# Autodesk Inventor assembly: center_4p_female
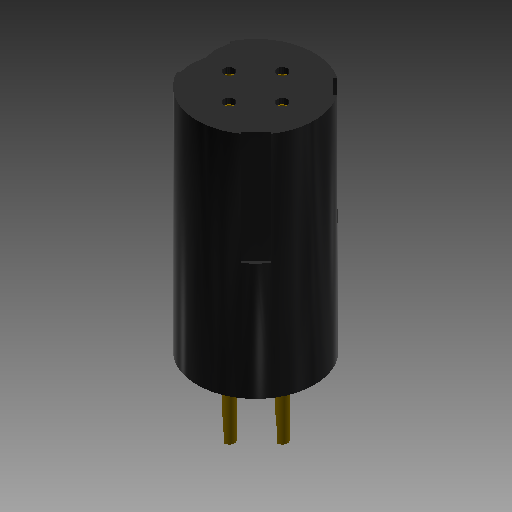
[picture p0: Inventor's stored thumbnail of the model, 512x512]
Saved by Autodesk Inventor 2018 (Build 220112000, 112)
## iProperties
Created: 2019-04-17
Part Number: center_4p_female
Document SubType Name: Assembly
Designer: ZEUSLAP
Author: ZEUSLAP
## Documents named in this file (3)
- C:\Users\ZEUSLAP\YandexDisk\Inventor\SP16 waterproof connector\parts\center_4p_female.iam
- C:\Users\ZEUSLAP\YandexDisk\Inventor\SP16 waterproof connector\parts\center_4p_female_body.ipt
- C:\Users\ZEUSLAP\YandexDisk\Inventor\SP16 waterproof connector\parts\pin_4p.ipt
## Components (5 placed, 2 different names)
1. center_2p_female_body:1 — Angle:1, Angle:2, Angle:3, Angle:4, Mate:1, Mate:2, Mate:3, Mate:4, Mate:5, Angle:5, Angle:6, Angle:7, Angle:8, Angle:9, Flush:4
2. pin_4p:1 — Angle:2, Flush:1, Flush:2, Mate:4, Angle:9
3. pin_4p:2 — Angle:3, Flush:2, Flush:3, Mate:3, Angle:8
4. pin_4p:3 — Angle:4, Flush:3, Mate:2, Angle:7
5. pin_4p:4 — Angle:1, Flush:1, Mate:1, Angle:6, Flush:4
## Relationships (18: Angle 9, Mate 5, Flush 4)
- Angle:1 (180 deg): center_2p_female_body:1 ↔ pin_4p:4
- Angle:2 (180 deg): center_2p_female_body:1 ↔ pin_4p:1
- Angle:3 (180 deg): center_2p_female_body:1 ↔ pin_4p:2
- Angle:4 (180 deg): center_2p_female_body:1 ↔ pin_4p:3
- Flush:1: pin_4p:1 ↔ pin_4p:4
- Flush:2: pin_4p:1 ↔ pin_4p:2
- Flush:3: pin_4p:2 ↔ pin_4p:3
- Mate:1: center_2p_female_body:1 ↔ pin_4p:4
- Mate:2: center_2p_female_body:1 ↔ pin_4p:3
- Mate:3: center_2p_female_body:1 ↔ pin_4p:2
- Mate:4: center_2p_female_body:1 ↔ pin_4p:1
- Mate:5: center_2p_female_body:1
- Angle:5 (180 deg): center_2p_female_body:1
- Angle:6 (90 deg): center_2p_female_body:1 ↔ pin_4p:4
- Angle:7 (270 deg): center_2p_female_body:1 ↔ pin_4p:3
- Angle:8 (270 deg): center_2p_female_body:1 ↔ pin_4p:2
- Angle:9 (270 deg): center_2p_female_body:1 ↔ pin_4p:1
- Flush:4 (6 mm): center_2p_female_body:1 ↔ pin_4p:4
